# Autodesk Inventor assembly: TH1-1001-CAM2
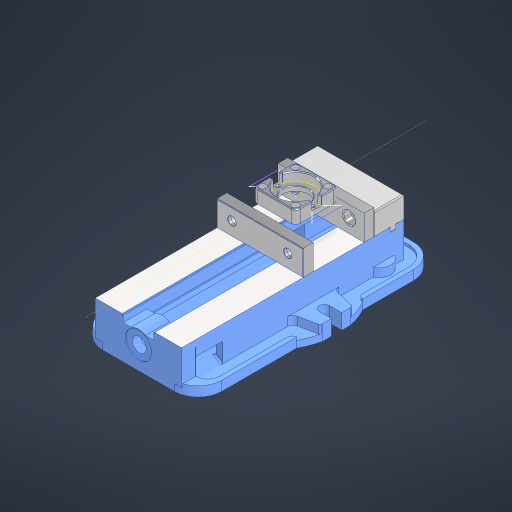
[picture p0: Inventor's stored thumbnail of the model, 512x512]
Saved by Autodesk Inventor 2024.3 (Build 283343000, 343)
## iProperties
Created: 2024-05-18
Part Number: TH1-1001-CAM2
Document SubType Name: Assembly
Designer: fablabadmin
Author: fablabadmin
## Documents named in this file (7)
- C:\Users\fablabadmin\Documents\_Benjamin_S\_3dCAD\HHVerkstad\ToolHolder1\_CAM\TH1-1001-CAM2.iam
- C:\Users\fablabadmin\Documents\_Benjamin_S\_3dCAD\_Config\KemmlerVise\OP1-KemmlerVise.iam
- C:\Users\fablabadmin\Documents\_Benjamin_S\_3dCAD\_Config\KemmlerVise\OP2-KemmlerVise.iam
- C:\Users\fablabadmin\Documents\Inventor\Content Center Files\R2024\en-US\StandardJaw\JawSTD-Aluminum 6061.ipt
- C:\Users\fablabadmin\Documents\_Benjamin_S\_3dCAD\HHVerkstad\ToolHolder1\TH1-001.ipt
- C:\Users\fablabadmin\Documents\_Benjamin_S\_3dCAD\HHVerkstad\ToolHolder1\_CAM\TH1-1001-CAM2-Stock.ipt
- C:\Users\fablabadmin\Documents\_Benjamin_S\_3dCAD\_Config\_CAM_SIM\FixtureParts\parallels3mm.xlsx
## Components (8 placed, 5 different names)
1. TH1-001:1 — Flush:5, Mate:10, Mate:11, Mate:12
2. TH1-1001-CAM2-Stock:1 — Flush:3, Flush:4, Flush:5, Mate:4, Mate:5, Mate:6
3. OP1-KemmlerVise:1 [sub-assembly] — Mate:1, Mate:2, Flush:1, Mate:3, Mate:6, Flush:6
4. JawStandard JawSTD-Aluminum 6061:1 — Mate:1, Flush:1, Flush:2, Mate:3, Mate:4
5. JawStandard JawSTD-Aluminum 6061:2 — Mate:2, Flush:2, Mate:5
6. OP2-KemmlerVise:1 [sub-assembly] — Mate:7, Mate:8, Flush:7, Mate:9, Mate:10, Mate:13
7. JawStandard JawSTD-Aluminum 6061:3 — Mate:8, Flush:8, Mate:12
8. JawStandard JawSTD-Aluminum 6061:4 — Mate:7, Flush:7, Flush:8, Mate:9, Mate:11
## Relationships (21: Mate 13, Flush 8)
- Mate:1: OP1-KemmlerVise:1 ↔ JawStandard JawSTD-Aluminum 6061:1
- Mate:2: OP1-KemmlerVise:1 ↔ JawStandard JawSTD-Aluminum 6061:2
- Flush:1: OP1-KemmlerVise:1 ↔ JawStandard JawSTD-Aluminum 6061:1
- Flush:2: JawStandard JawSTD-Aluminum 6061:1 ↔ JawStandard JawSTD-Aluminum 6061:2
- Mate:3: OP1-KemmlerVise:1 ↔ JawStandard JawSTD-Aluminum 6061:1
- Flush:3: TH1-1001-CAM2-Stock:1
- Flush:4: TH1-1001-CAM2-Stock:1
- Flush:5 (-1 mm): TH1-001:1 ↔ TH1-1001-CAM2-Stock:1
- Mate:4: TH1-1001-CAM2-Stock:1 ↔ JawStandard JawSTD-Aluminum 6061:1
- Mate:5: TH1-1001-CAM2-Stock:1 ↔ JawStandard JawSTD-Aluminum 6061:2
- Mate:6 (31 mm): TH1-1001-CAM2-Stock:1 ↔ OP1-KemmlerVise:1
- Flush:6: OP1-KemmlerVise:1
- Mate:7: OP2-KemmlerVise:1 ↔ JawStandard JawSTD-Aluminum 6061:4
- Mate:8: OP2-KemmlerVise:1 ↔ JawStandard JawSTD-Aluminum 6061:3
- Flush:7: OP2-KemmlerVise:1 ↔ JawStandard JawSTD-Aluminum 6061:4
- Flush:8: JawStandard JawSTD-Aluminum 6061:3 ↔ JawStandard JawSTD-Aluminum 6061:4
- Mate:9: OP2-KemmlerVise:1 ↔ JawStandard JawSTD-Aluminum 6061:4
- Mate:10 (28 mm): TH1-001:1 ↔ OP2-KemmlerVise:1
- Mate:11: TH1-001:1 ↔ JawStandard JawSTD-Aluminum 6061:4
- Mate:12: TH1-001:1 ↔ JawStandard JawSTD-Aluminum 6061:3
- Mate:13: OP2-KemmlerVise:1
## Named parameters: PRL13 = 13 mm, PRL16 = 16 mm, PRL19 = 19 mm, PRL22 = 22 mm, PRL28 = 28 mm, PRL31 = 31 mm, PRL35 = 35 mm, PRL38 = 38 mm, PRL41 = 41 mm
